# Autodesk Inventor assembly: Intake
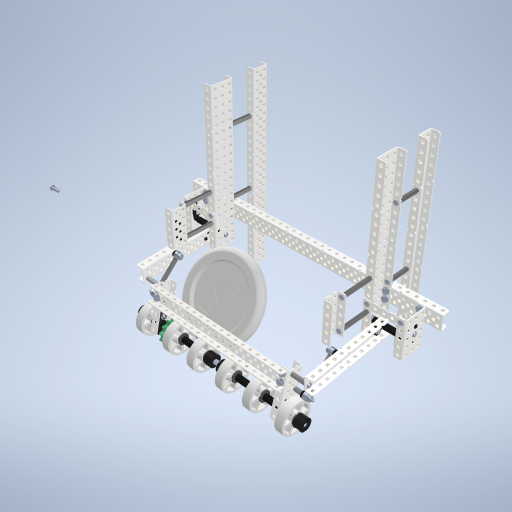
[picture p0: Inventor's stored thumbnail of the model, 512x512]
Saved by Autodesk Inventor 2023 (Build 270158000, 158)
## iProperties
Created: 2022-09-02
Part Number: Intake
Document SubType Name: Assembly
Designer: alex
Author: alex
## Documents named in this file (44)
- C:\Users\alex\Documents\GitHub\4067X_spin_up_cad\Mechanism\Intake.iam
- C:\Users\alex\Documents\GitHub\4067X_spin_up_cad\Library\Structure\Standoff\Standoff 1.00.ipt
- C:\Users\alex\Documents\GitHub\4067X_spin_up_cad\Library\Structure\Standoff.ipt
- C:\Users\alex\Documents\GitHub\4067X_spin_up_cad\Library\Structure\Standoff\Standoff 2.00.ipt
- C:\Users\alex\Documents\GitHub\4067X_spin_up_cad\Library\Structure\Hardware\Screw Steel - Star\SScrew Star Smooth .290.ipt
- C:\Users\alex\Documents\GitHub\4067X_spin_up_cad\Library\Structure\Hardware\Screw Steel - Star.ipt
- C:\Users\alex\Documents\GitHub\4067X_spin_up_cad\Library\Structure\Standoff\Standoff .50.ipt
- C:\Users\alex\Documents\GitHub\4067X_spin_up_cad\Library\Motion\Spacers\Spacer Nylon .375 OD.ipt
- C:\Users\alex\Documents\GitHub\4067X_spin_up_cad\Library\Structure\C-Channels\Aluminum 1x2x1\Alu C 1x2x1x6.ipt
- C:\Users\alex\Documents\GitHub\4067X_spin_up_cad\Library\Motion\Shaft HS\Shaft HS\Shaft HS 12.0 in.ipt
- C:\Users\alex\Documents\GitHub\4067X_spin_up_cad\Library\Motion\Shaft HS\Shaft HS.ipt
- C:\Users\alex\Documents\GitHub\4067X_spin_up_cad\Library\Motion\Spacers\Spacer Nylon .375 OD\NSpacer .375 OD x .125.ipt
- C:\Users\alex\Documents\GitHub\4067X_spin_up_cad\Library\Motion\Shaft Collar with Set Screw.ipt
- C:\Users\alex\Documents\GitHub\4067X_spin_up_cad\WithAdapter2Inch.iam
- C:\Users\alex\Documents\GitHub\4067X_spin_up_cad\Library\Motion\Shaft HS\HS Shaft Collar.ipt
- C:\Users\alex\Documents\GitHub\4067X_spin_up_cad\Library\Structure\Hardware\Screw Steel - Star\SScrew Star Smooth 1.250.ipt
- C:\Users\alex\Documents\GitHub\4067X_spin_up_cad\Library\Structure\Hardware\Nut Keps.ipt
- C:\Users\alex\Documents\GitHub\4067X_spin_up_cad\Library\Structure\Hardware\Screw Steel - Star\SScrew Star Smooth .625.ipt
- C:\Users\alex\Documents\GitHub\4067X_spin_up_cad\Library\Structure\C-Channels\Aluminum 1x2x1\Alu C 1x2x1x12.ipt
- C:\Users\alex\Documents\GitHub\4067X_spin_up_cad\Library\Motion\1-Post Bearing Flat Hex Retainer.ipt
- C:\Users\alex\Documents\GitHub\4067X_spin_up_cad\Library\Structure\Hardware\Screw Steel - Star\SScrew Star Smooth .375.ipt
- C:\Users\alex\Documents\GitHub\4067X_spin_up_cad\Library\Structure\Hardware\Nut Nylock.ipt
- C:\Users\alex\Documents\GitHub\4067X_spin_up_cad\Library\Structure\C-Channels\Aluminum 1x3x1\Alu C 1x3x1x20.ipt
- C:\Users\alex\Documents\GitHub\4067X_spin_up_cad\SpinUp\Disc.iam
- C:\Users\alex\Documents\GitHub\4067X_spin_up_cad\Library\Structure\C-Channels\Aluminum 1x3x1\Alu C 1x3x1x5.ipt
- C:\Users\alex\Documents\GitHub\4067X_spin_up_cad\Library\Structure\C-Channels\Aluminum 1x2x1\Alu C 1x2x1x35.ipt
- C:\Users\alex\Documents\GitHub\4067X_spin_up_cad\Library\Structure\Plates\Aluminum\VEX Plates\Alu Plate VEX 1x5.ipt
- C:\Users\alex\Documents\GitHub\4067X_spin_up_cad\Library\Structure\Hardware\Screw Steel - Star\SScrew Star Smooth 2.500.ipt
- C:\Users\alex\Documents\GitHub\4067X_spin_up_cad\Library\Motion\Spacers\Spacer Nylon .375 OD\NSpacer .375 OD x .375.ipt
- C:\Users\alex\Documents\GitHub\4067X_spin_up_cad\Library\Motion\Spacers\Washer Steel\SWasher .375 OD x .015625.ipt
- C:\Users\alex\Documents\GitHub\4067X_spin_up_cad\Library\Motion\Spacers\Washer Steel.ipt
- C:\Users\alex\Documents\GitHub\4067X_spin_up_cad\Library\Motion\Spacers\Spacer Nylon .375 OD\NSpacer .375 OD x .500.ipt
- C:\Users\alex\Documents\GitHub\4067X_spin_up_cad\Library\Structure\C-Channels\Aluminum 1x2x1\Alu C 1x2x1x25.ipt
- C:\Users\alex\Documents\GitHub\4067X_spin_up_cad\Library\Motion\Shaft HS\HS Bearing Flat.ipt
- C:\Users\alex\Documents\GitHub\4067X_spin_up_cad\Library\Motion\Shaft HS\HS Spacer\HSpacer .0625.ipt
- C:\Users\alex\Documents\GitHub\4067X_spin_up_cad\Library\Motion\Shaft HS\HS Spacer.ipt
- C:\Users\alex\Documents\GitHub\4067X_spin_up_cad\Library\Structure\Hardware\Screw Steel - Star\SScrew Star Smooth .500.ipt
- C:\Users\alex\Documents\GitHub\4067X_spin_up_cad\Library\Structure\Hardware\Nut Thin Nylock.ipt
- C:\Users\alex\Documents\GitHub\4067X_spin_up_cad\Library\Motion\Shaft HS\HS Spacer\HSpacer .5000.ipt
- C:\Users\alex\Documents\GitHub\4067X_spin_up_cad\Library\Motion\Shaft HS\HS Spacer\HSpacer .2500.ipt
- C:\Users\alex\Documents\GitHub\4067X_spin_up_cad\Library\Motion\Sprockets\HS 12T Sprocket, No Insert.ipt
- C:\Users\alex\Documents\GitHub\4067X_spin_up_cad\Library\Structure\C-Channels\Aluminum 1x2x1\Alu C 1x2x1x19.ipt
- C:\Users\alex\Documents\GitHub\4067X_spin_up_cad\Library\Structure\Hardware\Screw Steel - Star\SScrew Star Smooth .750.ipt
- C:\Users\alex\Documents\GitHub\4067X_spin_up_cad\Library\Structure\C-Channels\Aluminum 1x2x1\Alu C 1x2x1x5.ipt
## Components (158 placed, 37 different names)
1. Alu C 1x2x1x6:1 — Mate:2, Mate:3, Insert:39, Insert:40, Insert:48, Insert:50, Insert:167, Mate:19, Mate:21, Insert:168, Flush:3, Insert:210, Insert:211
2. Shaft HS 12.0 in:1 — Mate:2, Mate:5, Mate:6, Mate:9, Mate:10, Flush:1, Mate:20, Mate:23, Mate:25, Mate:26, Mate:28, Mate:29
3. NSpacer .375 OD x .125:1 — Insert:34, Insert:73
4. Shaft Collar with Set Screw:1 — Insert:34, Mate:4, Mate:7, Insert:53
5. Shaft Collar with Set Screw:2 — Mate:3, Mate:4, Insert:35, Insert:49
6. WithAdapter2Inch:1 [sub-assembly] — Mate:5, Mate:6, Mate:8, Mate:22
7. Standoff 2.00:12 — Insert:35, Mate:7
8. Standoff .50:14 — Insert:38, Insert:39
9. NSpacer .375 OD x .125:2 — Insert:38
10. Standoff 1.00:15 — Insert:40, Insert:71
11. HS Shaft Collar:1 — Mate:8, Mate:9, Mate:10, Flush:1
12. SScrew Star Smooth 1.250:13 — Insert:48
13. Nut Keps:1 — Insert:49
14. SScrew Star Smooth .290:14 — Insert:50
15. SScrew Star Smooth .290:15 — Insert:72
16. SScrew Star Smooth .625:16 — Insert:74
17. Nut Keps:2 — Insert:53
18. Alu C 1x2x1x12:1 — Insert:71, Insert:72, Insert:73, Insert:74, Insert:102, Mate:12, Insert:103, Mate:14, Flush:2
19. 1-Post Bearing Flat Hex Retainer:1 — Insert:102, Mate:12, Insert:104, Mate:13, Insert:121
20. SScrew Star Smooth .375:30 — Insert:103
21. Nut Nylock:1 — Insert:104
22. Alu C 1x3x1x20:1 — Mate:13, Mate:14, Insert:105, Insert:106, Insert:109, Insert:113, Insert:115, Insert:116, Insert:117, Insert:231, Insert:234, Insert:235, Insert:238, Insert:241
23. Alu C 1x3x1x5:1 — Insert:107, Insert:108, Insert:114, Insert:120, Mate:15, Insert:145, Insert:230, Insert:244, Insert:245
24. Alu C 1x2x1x35:1 — Insert:105, Insert:106, Insert:107, Insert:108, Insert:126, Insert:127, Insert:150, Insert:151, Insert:218, Insert:219, Insert:222, Insert:223, Insert:232, Insert:233, Insert:236, Insert:237
25. Standoff 1.00:16 — Insert:109, Insert:110
26. Standoff .50:17 — Insert:110, Insert:125
27. Standoff 1.00:18 — Insert:113
28. Standoff .50:19 — Insert:124
29. Alu Plate VEX 1x5:1 — Insert:114, Insert:115, Insert:228, Insert:229
30. SScrew Star Smooth 2.500:31 — Insert:116
31. Nut Keps:3 — Insert:117, Insert:118
32. NSpacer .375 OD x .375:3 — Insert:119
33. SWasher .375 OD x .015625:1 — Insert:118, Insert:119
34. 1-Post Bearing Flat Hex Retainer:2 — Insert:120, Mate:15, Insert:146
35. NSpacer .375 OD x .500:4 — Insert:121, Insert:122
36. NSpacer .375 OD x .500:5 — Insert:122, Insert:123
37. NSpacer .375 OD x .375:6 — Insert:123
38. Disc:1 [sub-assembly]
39. Alu C 1x2x1x25:1 — Insert:124, Insert:125, Insert:239, Insert:240
40. Alu C 1x3x1x20:2 — Insert:126, Insert:127, Insert:129, Insert:131, Insert:134, Insert:137, Insert:153, Mate:31, Insert:216, Insert:224, Insert:225, Insert:226, Insert:242, Insert:256, Insert:257
41. Standoff 1.00:20 — Insert:129
42. Standoff .50:21 — Insert:133
43. Standoff 1.00:22 — Insert:131
44. Standoff .50:23 — Insert:132
45. Alu C 1x2x1x25:2 — Insert:132, Insert:133, Insert:227, Insert:243
46. SScrew Star Smooth 2.500:32 — Insert:134, Mate:32
47. Nut Keps:4 — Insert:137
48. NSpacer .375 OD x .375:7
49. SWasher .375 OD x .015625:2
50. Alu C 1x2x1x12:2 — Insert:154, Insert:157, Flush:2, Insert:158, Insert:159, Mate:31, Mate:32
51. 1-Post Bearing Flat Hex Retainer:3 — Insert:144
52. SScrew Star Smooth .375:33
53. Nut Nylock:2
54. NSpacer .375 OD x .500:8 — Insert:144
55. NSpacer .375 OD x .500:9
56. NSpacer .375 OD x .375:10
57. SScrew Star Smooth .375:34 — Insert:145
58. Nut Nylock:3 — Insert:146
59. Alu C 1x3x1x5:2 — Insert:150, Insert:151, Insert:152, Insert:217, Insert:220, Insert:221
60. 1-Post Bearing Flat Hex Retainer:4
61. SScrew Star Smooth .375:35
62. Nut Nylock:4
63. Alu Plate VEX 1x5:2 — Insert:152, Insert:153, Insert:214, Insert:215
64. SScrew Star Smooth .625:36 — Insert:154
65. NSpacer .375 OD x .125:11 — Insert:157
66. Shaft Collar with Set Screw:3 — Insert:162
67. Nut Keps:5
68. SScrew Star Smooth .290:37 — Insert:158
69. Standoff 1.00:24 — Insert:159, Insert:160
70. Alu C 1x2x1x6:2 — Insert:160, Mate:18, Insert:164, Insert:165, Mate:24, Insert:171, Insert:172, Insert:173, Insert:199, Insert:200, Flush:3, Insert:205, Insert:206, Insert:207
71. Shaft Collar with Set Screw:4 — Mate:18, Insert:166
72. Standoff 2.00:25 — Insert:162
73. Standoff .50:26 — Insert:164
74. NSpacer .375 OD x .125:12
75. SScrew Star Smooth 1.250:38 — Insert:165
76. Nut Keps:6 — Insert:166
77. HS Bearing Flat:1 — Insert:167, Mate:19, Insert:169, Insert:188
78. HSpacer .0625:1 — Mate:20, Mate:21, Mate:22
79. SScrew Star Smooth .500:39 — Insert:168
80. Nut Thin Nylock:1 — Insert:169
81. HSpacer .0625:2 — Mate:23, Mate:24, Mate:27
82. WithAdapter2Inch:2 [sub-assembly] — Mate:25, Mate:26, Mate:27, Mate:30
83. HS Shaft Collar:2 — Mate:28, Mate:29, Mate:30
84. HS Bearing Flat:2 — Insert:171, Insert:172, Insert:189
85. Nut Thin Nylock:2
86. SScrew Star Smooth .500:40 — Insert:173
87. WithAdapter2Inch:3 [sub-assembly] — Insert:178, Insert:191
88. HSpacer .5000:5 — Insert:178, Insert:192
89. HSpacer .5000:6 — Insert:192, Insert:193
90. WithAdapter2Inch:4 [sub-assembly] — Insert:194, Insert:197
91. WithAdapter2Inch:5 [sub-assembly] — Insert:196, Insert:198
92. HSpacer .5000:9 — Insert:195
93. HSpacer .5000:10 — Insert:187
94. WithAdapter2Inch:6 [sub-assembly] — Insert:187
95. HSpacer .5000:11
96. HSpacer .5000:12 — Insert:188
97. HS 12T Sprocket, No Insert:1 — Insert:190, Insert:191
98. HSpacer .5000:13 — Insert:189, Insert:190
99. HSpacer .2500:14 — Insert:193, Insert:194
100. HSpacer .2500:15 — Insert:195, Insert:196
101. HS Shaft Collar:3 — Insert:197
102. HS Shaft Collar:4 — Insert:198
103. Alu C 1x2x1x19:1 — Insert:199, Insert:200, Insert:208, Insert:209, Insert:212, Insert:213
104. SScrew Star Smooth .290:45 — Insert:205
105. SScrew Star Smooth .290:46 — Insert:206
106. SScrew Star Smooth .290:47 — Insert:207
107. Nut Keps:7 — Insert:208
108. Nut Keps:8 — Insert:209
109. SScrew Star Smooth .290:48 — Insert:210
110. SScrew Star Smooth .290:49 — Insert:211
111. Nut Keps:9 — Insert:212
112. Nut Keps:10 — Insert:213
113. SScrew Star Smooth .290:50 — Insert:214
114. SScrew Star Smooth .290:51 — Insert:215
115. Nut Keps:11 — Insert:216
116. Nut Keps:12 — Insert:217
117. SScrew Star Smooth .290:52 — Insert:218
118. SScrew Star Smooth .290:53 — Insert:219
119. Nut Keps:13 — Insert:220
120. Nut Keps:14 — Insert:221
121. SScrew Star Smooth .290:54 — Insert:222
122. SScrew Star Smooth .290:55 — Insert:223
123. Nut Keps:15 — Insert:224
124. Nut Keps:16 — Insert:225
125. SScrew Star Smooth .290:56 — Insert:226
126. SScrew Star Smooth .750:57 — Insert:227
127. SScrew Star Smooth .290:58 — Insert:228
128. SScrew Star Smooth .290:59 — Insert:229
129. Nut Keps:17 — Insert:230
130. Nut Keps:18 — Insert:231
131. SScrew Star Smooth .290:60 — Insert:232
132. SScrew Star Smooth .290:61 — Insert:233
133. Nut Keps:19 — Insert:234
134. Nut Keps:20 — Insert:235
135. SScrew Star Smooth .290:62 — Insert:236
136. SScrew Star Smooth .290:63 — Insert:237
137. SScrew Star Smooth .290:64 — Insert:238
138. SScrew Star Smooth .750:65 — Insert:239
139. SScrew Star Smooth .750:66 — Insert:240
140. SScrew Star Smooth .290:67 — Insert:241
141. SScrew Star Smooth .290:68 — Insert:242
142. SScrew Star Smooth .750:69 — Insert:243
143. Nut Keps:21 — Insert:244
144. Nut Keps:22 — Insert:245
145. Standoff 2.00:27 — Insert:249
146. Standoff 2.00:28 — Insert:248
147. Alu C 1x2x1x5:1 — Insert:248, Insert:249, Insert:250, Insert:251
148. SScrew Star Smooth .290:70 — Insert:250
149. SScrew Star Smooth .290:71 — Insert:251
150. Standoff 2.00:29 — Insert:256
151. Standoff 2.00:30 — Insert:257
152. Alu C 1x2x1x5:2 — Insert:259, Mate:33
153. SScrew Star Smooth .290:72
154. SScrew Star Smooth .290:73
155. HS Bearing Flat:3 — Insert:259, Mate:33, Insert:260
156. Nut Thin Nylock:3
157. SScrew Star Smooth .500:74
158. Nut Thin Nylock:4 — Insert:260
## Relationships (191: Insert 157, Mate 31, Flush 3)
- Mate:2: Alu C 1x2x1x6:1 ↔ Shaft HS 12.0 in:1
- Insert:34: NSpacer .375 OD x .125:1 ↔ Shaft Collar with Set Screw:1
- Mate:3: Alu C 1x2x1x6:1 ↔ Shaft Collar with Set Screw:2
- Mate:4: Shaft Collar with Set Screw:1 ↔ Shaft Collar with Set Screw:2
- Mate:5: Shaft HS 12.0 in:1 ↔ WithAdapter2Inch:1
- Mate:6: Shaft HS 12.0 in:1 ↔ WithAdapter2Inch:1
- Insert:35 (-0.3556 mm): Shaft Collar with Set Screw:2 ↔ Standoff 2.00:12
- Mate:7 (-0.3556 mm): Shaft Collar with Set Screw:1 ↔ Standoff 2.00:12
- Insert:38: Standoff .50:14 ↔ NSpacer .375 OD x .125:2
- Insert:39: Alu C 1x2x1x6:1 ↔ Standoff .50:14
- Insert:40: Alu C 1x2x1x6:1 ↔ Standoff 1.00:15
- Mate:8: WithAdapter2Inch:1 ↔ HS Shaft Collar:1
- Mate:9: Shaft HS 12.0 in:1 ↔ HS Shaft Collar:1
- Mate:10: Shaft HS 12.0 in:1 ↔ HS Shaft Collar:1
- Flush:1 (1.27 mm): Shaft HS 12.0 in:1 ↔ HS Shaft Collar:1
- Insert:48: Alu C 1x2x1x6:1 ↔ SScrew Star Smooth 1.250:13
- Insert:49: Shaft Collar with Set Screw:2 ↔ Nut Keps:1
- Insert:50: Alu C 1x2x1x6:1 ↔ SScrew Star Smooth .290:14
- Insert:53: Shaft Collar with Set Screw:1 ↔ Nut Keps:2
- Insert:71: Standoff 1.00:15 ↔ Alu C 1x2x1x12:1
- Insert:72: SScrew Star Smooth .290:15 ↔ Alu C 1x2x1x12:1
- Insert:73: NSpacer .375 OD x .125:1 ↔ Alu C 1x2x1x12:1
- Insert:74: SScrew Star Smooth .625:16 ↔ Alu C 1x2x1x12:1
- Insert:102: Alu C 1x2x1x12:1 ↔ 1-Post Bearing Flat Hex Retainer:1
- Mate:12: Alu C 1x2x1x12:1 ↔ 1-Post Bearing Flat Hex Retainer:1
- Insert:103: Alu C 1x2x1x12:1 ↔ SScrew Star Smooth .375:30
- Insert:104: 1-Post Bearing Flat Hex Retainer:1 ↔ Nut Nylock:1
- Mate:13: 1-Post Bearing Flat Hex Retainer:1 ↔ Alu C 1x3x1x20:1
- Mate:14 (13.6398 mm): Alu C 1x2x1x12:1 ↔ Alu C 1x3x1x20:1
- Insert:105: Alu C 1x3x1x20:1 ↔ Alu C 1x2x1x35:1
- Insert:106: Alu C 1x3x1x20:1 ↔ Alu C 1x2x1x35:1
- Insert:107: Alu C 1x3x1x5:1 ↔ Alu C 1x2x1x35:1
- Insert:108: Alu C 1x3x1x5:1 ↔ Alu C 1x2x1x35:1
- Insert:109: Alu C 1x3x1x20:1 ↔ Standoff 1.00:16
- Insert:110: Standoff 1.00:16 ↔ Standoff .50:17
- [Insert]: Standoff 1.00:18 ↔ Standoff .50:19
- Insert:113: Alu C 1x3x1x20:1 ↔ Standoff 1.00:18
- Insert:114: Alu C 1x3x1x5:1 ↔ Alu Plate VEX 1x5:1
- Insert:115: Alu C 1x3x1x20:1 ↔ Alu Plate VEX 1x5:1
- Insert:116: Alu C 1x3x1x20:1 ↔ SScrew Star Smooth 2.500:31
- Insert:117: Alu C 1x3x1x20:1 ↔ Nut Keps:3
- Insert:118: Nut Keps:3 ↔ SWasher .375 OD x .015625:1
- Insert:119: NSpacer .375 OD x .375:3 ↔ SWasher .375 OD x .015625:1
- Insert:120: Alu C 1x3x1x5:1 ↔ 1-Post Bearing Flat Hex Retainer:2
- Mate:15: Alu C 1x3x1x5:1 ↔ 1-Post Bearing Flat Hex Retainer:2
- Insert:121: 1-Post Bearing Flat Hex Retainer:1 ↔ NSpacer .375 OD x .500:4
- Insert:122: NSpacer .375 OD x .500:4 ↔ NSpacer .375 OD x .500:5
- Insert:123: NSpacer .375 OD x .500:5 ↔ NSpacer .375 OD x .375:6
- Insert:124: Standoff .50:19 ↔ Alu C 1x2x1x25:1
- Insert:125: Standoff .50:17 ↔ Alu C 1x2x1x25:1
- Insert:126: Alu C 1x2x1x35:1 ↔ Alu C 1x3x1x20:2
- Insert:127: Alu C 1x2x1x35:1 ↔ Alu C 1x3x1x20:2
- [Insert]: Standoff 1.00:20 ↔ Standoff .50:21
- Insert:129: Alu C 1x3x1x20:2 ↔ Standoff 1.00:20
- [Insert]: Standoff 1.00:22 ↔ Standoff .50:23
- Insert:131: Alu C 1x3x1x20:2 ↔ Standoff 1.00:22
- Insert:132: Standoff .50:23 ↔ Alu C 1x2x1x25:2
- Insert:133: Standoff .50:21 ↔ Alu C 1x2x1x25:2
- Insert:134: Alu C 1x3x1x20:2 ↔ SScrew Star Smooth 2.500:32
- [Insert]: Nut Keps:4 ↔ SWasher .375 OD x .015625:2
- [Insert]: NSpacer .375 OD x .375:7 ↔ SWasher .375 OD x .015625:2
- Insert:137: Alu C 1x3x1x20:2 ↔ Nut Keps:4
- [Insert]: Alu C 1x2x1x12:2 ↔ 1-Post Bearing Flat Hex Retainer:3
- [Mate]: Alu C 1x2x1x12:2 ↔ 1-Post Bearing Flat Hex Retainer:3
- [Insert]: Alu C 1x2x1x12:2 ↔ SScrew Star Smooth .375:33
- [Insert]: 1-Post Bearing Flat Hex Retainer:3 ↔ Nut Nylock:2
- [Insert]: NSpacer .375 OD x .500:8 ↔ NSpacer .375 OD x .500:9
- [Insert]: NSpacer .375 OD x .500:9 ↔ NSpacer .375 OD x .375:10
- Insert:144: 1-Post Bearing Flat Hex Retainer:3 ↔ NSpacer .375 OD x .500:8
- Insert:145: Alu C 1x3x1x5:1 ↔ SScrew Star Smooth .375:34
- Insert:146: 1-Post Bearing Flat Hex Retainer:2 ↔ Nut Nylock:3
- [Insert]: Alu C 1x3x1x5:2 ↔ 1-Post Bearing Flat Hex Retainer:4
- [Mate]: Alu C 1x3x1x5:2 ↔ 1-Post Bearing Flat Hex Retainer:4
- [Insert]: Alu C 1x3x1x5:2 ↔ SScrew Star Smooth .375:35
- [Insert]: 1-Post Bearing Flat Hex Retainer:4 ↔ Nut Nylock:4
- Insert:150: Alu C 1x2x1x35:1 ↔ Alu C 1x3x1x5:2
- Insert:151: Alu C 1x2x1x35:1 ↔ Alu C 1x3x1x5:2
- Insert:152: Alu C 1x3x1x5:2 ↔ Alu Plate VEX 1x5:2
- Insert:153: Alu C 1x3x1x20:2 ↔ Alu Plate VEX 1x5:2
- Insert:154: Alu C 1x2x1x12:2 ↔ SScrew Star Smooth .625:36
- [Insert]: NSpacer .375 OD x .125:11 ↔ Shaft Collar with Set Screw:3
- [Insert]: Shaft Collar with Set Screw:3 ↔ Nut Keps:5
- Insert:157: Alu C 1x2x1x12:2 ↔ NSpacer .375 OD x .125:11
- Flush:2: Alu C 1x2x1x12:1 ↔ Alu C 1x2x1x12:2
- Insert:158: Alu C 1x2x1x12:2 ↔ SScrew Star Smooth .290:37
- Insert:159: Alu C 1x2x1x12:2 ↔ Standoff 1.00:24
- Insert:160: Standoff 1.00:24 ↔ Alu C 1x2x1x6:2
- [Insert] (-0.3556 mm): Shaft Collar with Set Screw:4 ↔ Standoff 2.00:25
- Insert:162 (-0.3556 mm): Shaft Collar with Set Screw:3 ↔ Standoff 2.00:25
- Mate:18: Alu C 1x2x1x6:2 ↔ Shaft Collar with Set Screw:4
- [Insert]: Standoff .50:26 ↔ NSpacer .375 OD x .125:12
- Insert:164: Alu C 1x2x1x6:2 ↔ Standoff .50:26
- Insert:165: Alu C 1x2x1x6:2 ↔ SScrew Star Smooth 1.250:38
- Insert:166: Shaft Collar with Set Screw:4 ↔ Nut Keps:6
- Insert:167: Alu C 1x2x1x6:1 ↔ HS Bearing Flat:1
- Mate:19: Alu C 1x2x1x6:1 ↔ HS Bearing Flat:1
- Mate:20: Shaft HS 12.0 in:1 ↔ HSpacer .0625:1
- Mate:21: Alu C 1x2x1x6:1 ↔ HSpacer .0625:1
- Mate:22: WithAdapter2Inch:1 ↔ HSpacer .0625:1
- Insert:168: Alu C 1x2x1x6:1 ↔ SScrew Star Smooth .500:39
- Insert:169: HS Bearing Flat:1 ↔ Nut Thin Nylock:1
- Mate:23: Shaft HS 12.0 in:1 ↔ HSpacer .0625:2
- Mate:24: Alu C 1x2x1x6:2 ↔ HSpacer .0625:2
- Mate:25: Shaft HS 12.0 in:1 ↔ WithAdapter2Inch:2
- Mate:26: Shaft HS 12.0 in:1 ↔ WithAdapter2Inch:2
- Mate:27: HSpacer .0625:2 ↔ WithAdapter2Inch:2
- Mate:28: Shaft HS 12.0 in:1 ↔ HS Shaft Collar:2
- Mate:29: Shaft HS 12.0 in:1 ↔ HS Shaft Collar:2
- Mate:30: WithAdapter2Inch:2 ↔ HS Shaft Collar:2
- [Insert]: HS Bearing Flat:2 ↔ Nut Thin Nylock:2
- Insert:171: Alu C 1x2x1x6:2 ↔ HS Bearing Flat:2
- Insert:172: Alu C 1x2x1x6:2 ↔ HS Bearing Flat:2
- Insert:173: Alu C 1x2x1x6:2 ↔ SScrew Star Smooth .500:40
- Insert:178: WithAdapter2Inch:3 ↔ HSpacer .5000:5
- [Insert]: HSpacer .5000:9 ↔ HSpacer .5000:10
- [Insert]: HSpacer .5000:11 ↔ HSpacer .5000:12
- [Insert]: WithAdapter2Inch:6 ↔ HSpacer .5000:11
- Insert:187: HSpacer .5000:10 ↔ WithAdapter2Inch:6
- Insert:188: HS Bearing Flat:1 ↔ HSpacer .5000:12
- Insert:189: HS Bearing Flat:2 ↔ HSpacer .5000:13
- Insert:190: HS 12T Sprocket, No Insert:1 ↔ HSpacer .5000:13
- Insert:191: WithAdapter2Inch:3 ↔ HS 12T Sprocket, No Insert:1
- Insert:192: HSpacer .5000:5 ↔ HSpacer .5000:6
- Insert:193: HSpacer .5000:6 ↔ HSpacer .2500:14
- Insert:194: WithAdapter2Inch:4 ↔ HSpacer .2500:14
- Insert:195: HSpacer .5000:9 ↔ HSpacer .2500:15
- Insert:196: WithAdapter2Inch:5 ↔ HSpacer .2500:15
- Insert:197: WithAdapter2Inch:4 ↔ HS Shaft Collar:3
- Insert:198: WithAdapter2Inch:5 ↔ HS Shaft Collar:4
- Mate:31 (13.6398 mm): Alu C 1x3x1x20:2 ↔ Alu C 1x2x1x12:2
- Mate:32: SScrew Star Smooth 2.500:32 ↔ Alu C 1x2x1x12:2
- Insert:199: Alu C 1x2x1x6:2 ↔ Alu C 1x2x1x19:1
- Insert:200: Alu C 1x2x1x6:2 ↔ Alu C 1x2x1x19:1
- Flush:3: Alu C 1x2x1x6:1 ↔ Alu C 1x2x1x6:2
- Insert:205: Alu C 1x2x1x6:2 ↔ SScrew Star Smooth .290:45
- Insert:206: Alu C 1x2x1x6:2 ↔ SScrew Star Smooth .290:46
- Insert:207: Alu C 1x2x1x6:2 ↔ SScrew Star Smooth .290:47
- Insert:208: Alu C 1x2x1x19:1 ↔ Nut Keps:7
- Insert:209: Alu C 1x2x1x19:1 ↔ Nut Keps:8
- Insert:210: Alu C 1x2x1x6:1 ↔ SScrew Star Smooth .290:48
- Insert:211: Alu C 1x2x1x6:1 ↔ SScrew Star Smooth .290:49
- Insert:212: Alu C 1x2x1x19:1 ↔ Nut Keps:9
- Insert:213: Alu C 1x2x1x19:1 ↔ Nut Keps:10
- Insert:214: Alu Plate VEX 1x5:2 ↔ SScrew Star Smooth .290:50
- Insert:215: Alu Plate VEX 1x5:2 ↔ SScrew Star Smooth .290:51
- Insert:216: Alu C 1x3x1x20:2 ↔ Nut Keps:11
- Insert:217: Alu C 1x3x1x5:2 ↔ Nut Keps:12
- Insert:218: Alu C 1x2x1x35:1 ↔ SScrew Star Smooth .290:52
- Insert:219: Alu C 1x2x1x35:1 ↔ SScrew Star Smooth .290:53
- Insert:220: Alu C 1x3x1x5:2 ↔ Nut Keps:13
- Insert:221: Alu C 1x3x1x5:2 ↔ Nut Keps:14
- Insert:222: Alu C 1x2x1x35:1 ↔ SScrew Star Smooth .290:54
- Insert:223: Alu C 1x2x1x35:1 ↔ SScrew Star Smooth .290:55
- Insert:224: Alu C 1x3x1x20:2 ↔ Nut Keps:15
- Insert:225: Alu C 1x3x1x20:2 ↔ Nut Keps:16
- Insert:226: Alu C 1x3x1x20:2 ↔ SScrew Star Smooth .290:56
- Insert:227: Alu C 1x2x1x25:2 ↔ SScrew Star Smooth .750:57
- Insert:228: Alu Plate VEX 1x5:1 ↔ SScrew Star Smooth .290:58
- Insert:229: Alu Plate VEX 1x5:1 ↔ SScrew Star Smooth .290:59
- Insert:230: Alu C 1x3x1x5:1 ↔ Nut Keps:17
- Insert:231: Alu C 1x3x1x20:1 ↔ Nut Keps:18
- Insert:232: Alu C 1x2x1x35:1 ↔ SScrew Star Smooth .290:60
- Insert:233: Alu C 1x2x1x35:1 ↔ SScrew Star Smooth .290:61
- Insert:234: Alu C 1x3x1x20:1 ↔ Nut Keps:19
- Insert:235: Alu C 1x3x1x20:1 ↔ Nut Keps:20
- Insert:236: Alu C 1x2x1x35:1 ↔ SScrew Star Smooth .290:62
- Insert:237: Alu C 1x2x1x35:1 ↔ SScrew Star Smooth .290:63
- Insert:238: Alu C 1x3x1x20:1 ↔ SScrew Star Smooth .290:64
- Insert:239: Alu C 1x2x1x25:1 ↔ SScrew Star Smooth .750:65
- Insert:240: Alu C 1x2x1x25:1 ↔ SScrew Star Smooth .750:66
- Insert:241: Alu C 1x3x1x20:1 ↔ SScrew Star Smooth .290:67
- Insert:242: Alu C 1x3x1x20:2 ↔ SScrew Star Smooth .290:68
- Insert:243: Alu C 1x2x1x25:2 ↔ SScrew Star Smooth .750:69
- Insert:244: Alu C 1x3x1x5:1 ↔ Nut Keps:21
- Insert:245: Alu C 1x3x1x5:1 ↔ Nut Keps:22
- [Insert]: Alu C 1x3x1x20:1 ↔ Standoff 2.00:27
- [Insert]: Alu C 1x3x1x20:1 ↔ Standoff 2.00:28
- Insert:248: Standoff 2.00:28 ↔ Alu C 1x2x1x5:1
- Insert:249: Standoff 2.00:27 ↔ Alu C 1x2x1x5:1
- Insert:250: Alu C 1x2x1x5:1 ↔ SScrew Star Smooth .290:70
- Insert:251: Alu C 1x2x1x5:1 ↔ SScrew Star Smooth .290:71
- [Insert]: Standoff 2.00:30 ↔ Alu C 1x2x1x5:2
- [Insert]: Standoff 2.00:29 ↔ Alu C 1x2x1x5:2
- [Insert]: Alu C 1x2x1x5:2 ↔ SScrew Star Smooth .290:72
- [Insert]: Alu C 1x2x1x5:2 ↔ SScrew Star Smooth .290:73
- Insert:256: Alu C 1x3x1x20:2 ↔ Standoff 2.00:29
- Insert:257: Alu C 1x3x1x20:2 ↔ Standoff 2.00:30
- [Insert]: HS Bearing Flat:3 ↔ Nut Thin Nylock:3
- Insert:259: Alu C 1x2x1x5:2 ↔ HS Bearing Flat:3
- Mate:33: Alu C 1x2x1x5:2 ↔ HS Bearing Flat:3
- Insert:260: HS Bearing Flat:3 ↔ Nut Thin Nylock:4
## Named parameters: d171_d169 = 0 mm, d195_d169 = 0 mm, d197_d195_d169 = 0 mm, d202_d181 = 0 mm, d203_d182 = 0 mm, d205_d144 = 0 mm, d206_d145 = 0 mm, d207_d146 = 0 mm, d208_d147 = 0 mm, d210_d188 = 0 mm, d211_d189 = 0 mm, d215_d185 = 0 mm, d216_d186 = 0 mm, d217_d213 = 0 mm, d218_d214 = 0 mm, d224_d43 = 0 mm, d225_d78 = 0 mm, d231_d48 = -0.3556 mm, d234_d52 = 0 mm, d253_d244 = 0 mm, d265_d262_d260_d258 = 0 mm, d268_d262_d260_d258 = 0 mm, d269_d263_d261 = 0 mm, d351_d348 = 0 mm, d352_d349 = 0 mm, d353_d350 = 0 mm, d354_d347 = 0 mm, d357_d253_d244 = 0 mm
